# Autodesk Inventor assembly: 5 Support Compartment Model 1
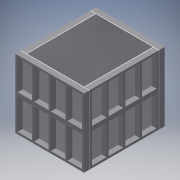
[picture p0: Inventor's stored thumbnail of the model, 180x180]
Saved by Autodesk Inventor 2017 (Build 210142000, 142)
## iProperties
Created: 2017-05-25
Part Number: 5 Support Compartment Model 1
Document SubType Name: Assembly
Designer: cas7
Author: cas7
## Documents named in this file (5)
- C:\Users\Public\Documents\Autodesk\.desktop-connect\.docstore\guided-tutorial-plugin\INVNTOR\5 Support Compartment Model 1.iam
- C:\Users\Public\Documents\Autodesk\.desktop-connect\.docstore\guided-tutorial-plugin\INVNTOR\2017\ENU\552100320579484105\TutorialModelPath\48in 2x4.ipt
- C:\Users\Public\Documents\Autodesk\.desktop-connect\.docstore\guided-tutorial-plugin\INVNTOR\2017\ENU\552100320579484105\TutorialModelPath\21in 2x4.ipt
- C:\Users\Public\Documents\Autodesk\.desktop-connect\.docstore\guided-tutorial-plugin\INVNTOR\2017\ENU\552100320579484105\TutorialModelPath\4x2 Gyp Board.ipt
- C:\Users\Public\Documents\Autodesk\.desktop-connect\.docstore\guided-tutorial-plugin\INVNTOR\5 Support Model.iam
## Components (22 placed, 3 different names)
1. 5 Support Model:1 [sub-assembly] — Mate:19, Mate:20, Mate:39, Mate:40, Mate:68
2. 5 Support Model:2 [sub-assembly] — Mate:19, Mate:20, Mate:41
3. 5 Support Model:3 [sub-assembly] — Mate:41, Mate:42
4. 4ft 2x4:8
5. 4ft 2x4:9 — Mate:42
6. 4ft 2x4:10 — Mate:39
7. 4ft 2x4:11 — Mate:40, Mate:67
8. 4ft 2x4:12
9. 4ft 2x4:13
10. 4ft 2x4:14
11. 4x2 Gyp Board:2
12. 5 Support Model:4 [sub-assembly] — Mate:68
13. 5 Support Model:5 [sub-assembly]
14. 5 Support Model:6 [sub-assembly]
15. 4ft 2x4:15 — Mate:67
16. 4ft 2x4:16
17. 4ft 2x4:17
18. 4ft 2x4:18
19. 4ft 2x4:19
20. 4ft 2x4:20
21. 4ft 2x4:21
22. 4x2 Gyp Board:3
## Relationships (50: Mate 50)
- Mate:19: 5 Support Model:1 ↔ 5 Support Model:2
- Mate:20: 5 Support Model:1 ↔ 5 Support Model:2
- [Mate]: 4ft 2x4:8 ↔ 4ft 2x4:9
- [Mate]: 4ft 2x4:8 ↔ 4ft 2x4:9
- [Mate]: 4ft 2x4:8 ↔ 4ft 2x4:9
- [Mate]: 4ft 2x4:8 ↔ 4ft 2x4:10
- [Mate]: 4ft 2x4:9 ↔ 4ft 2x4:11
- [Mate]: 4ft 2x4:9 ↔ 4ft 2x4:11
- [Mate]: 4ft 2x4:8 ↔ 4ft 2x4:12
- [Mate]: 4ft 2x4:8 ↔ 4ft 2x4:13
- [Mate]: 4ft 2x4:8 ↔ 4ft 2x4:14
- [Mate]: 4ft 2x4:8 ↔ 4ft 2x4:12
- [Mate]: 4ft 2x4:8 ↔ 4ft 2x4:13
- [Mate]: 4ft 2x4:8 ↔ 4ft 2x4:14
- [Mate]: 4ft 2x4:10 ↔ 4x2 Gyp Board:2
- [Mate]: 4ft 2x4:11 ↔ 4x2 Gyp Board:2
- [Mate]: 4ft 2x4:11 ↔ 4ft 2x4:13
- [Mate]: 4ft 2x4:11 ↔ 4ft 2x4:14
- [Mate]: 4ft 2x4:11 ↔ 4ft 2x4:12
- [Mate]: 4ft 2x4:10 ↔ 4ft 2x4:11
- Mate:39: 5 Support Model:1 ↔ 4ft 2x4:10
- Mate:40: 5 Support Model:1 ↔ 4ft 2x4:11
- Mate:41: 5 Support Model:2 ↔ 5 Support Model:3
- Mate:42: 5 Support Model:3 ↔ 4ft 2x4:9
- [Mate]: 5 Support Model:4 ↔ 5 Support Model:5
- [Mate]: 5 Support Model:4 ↔ 5 Support Model:5
- [Mate]: 4ft 2x4:15 ↔ 4ft 2x4:16
- [Mate]: 4ft 2x4:15 ↔ 4ft 2x4:16
- [Mate]: 4ft 2x4:15 ↔ 4ft 2x4:16
- [Mate]: 4ft 2x4:15 ↔ 4ft 2x4:17
- [Mate]: 4ft 2x4:16 ↔ 4ft 2x4:18
- [Mate]: 4ft 2x4:16 ↔ 4ft 2x4:18
- [Mate]: 4ft 2x4:15 ↔ 4ft 2x4:19
- [Mate]: 4ft 2x4:15 ↔ 4ft 2x4:20
- [Mate]: 4ft 2x4:15 ↔ 4ft 2x4:21
- [Mate]: 4ft 2x4:15 ↔ 4ft 2x4:19
- [Mate]: 4ft 2x4:15 ↔ 4ft 2x4:20
- [Mate]: 4ft 2x4:15 ↔ 4ft 2x4:21
- [Mate]: 4ft 2x4:17 ↔ 4x2 Gyp Board:3
- [Mate]: 4ft 2x4:18 ↔ 4x2 Gyp Board:3
- [Mate]: 4ft 2x4:18 ↔ 4ft 2x4:20
- [Mate]: 4ft 2x4:18 ↔ 4ft 2x4:21
- [Mate]: 4ft 2x4:18 ↔ 4ft 2x4:19
- [Mate]: 4ft 2x4:17 ↔ 4ft 2x4:18
- [Mate]: 5 Support Model:4 ↔ 4ft 2x4:17
- [Mate]: 5 Support Model:4 ↔ 4ft 2x4:18
- [Mate]: 5 Support Model:5 ↔ 5 Support Model:6
- [Mate]: 5 Support Model:6 ↔ 4ft 2x4:16
- Mate:67: 4ft 2x4:11 ↔ 4ft 2x4:15
- Mate:68: 5 Support Model:1 ↔ 5 Support Model:4
## Named parameters: d26_d0 = 0 mm, d27_d1 = 0 mm, d28_d2 = 0 mm, d29_d3_d8 = 0 mm, d30_d4_d10 = 0 mm, d31_d5_d11 = 0 mm, d32_d6_d12 = 0 mm, d33_d7_d13 = 0 mm, d34_d8_d14 = 0 mm, d35_d9_d15 = 0 mm, d36_d10_d16 = 0 mm, d37_d11_d17 = 0 mm, d38_d18 = 0 mm, d39_d19 = 0 mm, d40_d20 = 0 mm, d41_d21 = 0 mm, d42_d22 = 0 mm, d43_d23 = 0 mm, d48_d24 = 0 mm, d49_d25 = 0 mm, d50_d26_d0 = 0 mm, d51_d27_d1 = 0 mm, d52_d28_d2 = 0 mm, d53_d29_d3_d8 = 0 mm, d54_d30_d4_d10 = 0 mm, d55_d31_d5_d11 = 0 mm, d56_d32_d6_d12 = 0 mm, d57_d33_d7_d13 = 0 mm, d58_d34_d8_d14 = 0 mm, d59_d35_d9_d15 = 0 mm, d60_d36_d10_d16 = 0 mm, d61_d37_d11_d17 = 0 mm, d62_d38_d18 = 0 mm, d63_d39_d19 = 0 mm, d64_d40_d20 = 0 mm, d65_d41_d21 = 0 mm, d66_d42_d22 = 0 mm, d67_d43_d23 = 0 mm, d68_d44 = 0 mm, d69_d45 = 0 mm, d70_d46 = 0 mm, d71_d47 = 0 mm
